# Autodesk Inventor assembly: Flange_tube
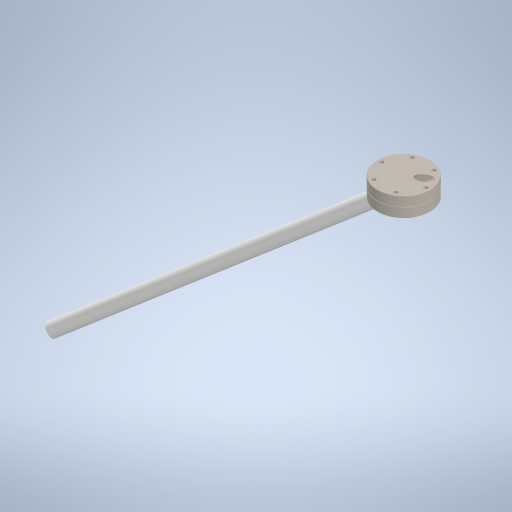
[picture p0: Inventor's stored thumbnail of the model, 512x512]
Saved by Autodesk Inventor 2024 (Build 280153000, 153)
## iProperties
Created: 2024-11-06
Part Number: Flange_tube
Document SubType Name: Assembly
Designer: Andreas Weber
Author: Andreas Weber
## Documents named in this file (4)
- C:\Users\Andreas Weber\Desktop\Upload for Github\Flange_tube.iam
- C:\Users\Andreas Weber\Desktop\Upload for Github\blank_flange_CF40.ipt
- C:\Users\Andreas Weber\Desktop\Upload for Github\blank_flange_thread_CF40.ipt
- C:\Users\Andreas Weber\Desktop\Upload for Github\tube_Brewster_angle.ipt
## Components (3 placed, 3 different names)
1. blank_flange_CF40:1 — Drehbar:1, Verschiebbar:1
2. blank_flange_thread_CF40:1 — Drehbar:1
3. tube_Brewster_angle:1 — Verschiebbar:1
## Relationships (2: RevoluteJoint 1, TranslationJoint 1)
- Drehbar:1 [RevoluteJoint]: blank_flange_CF40:1 ↔ blank_flange_thread_CF40:1
- Verschiebbar:1 [TranslationJoint]: blank_flange_CF40:1 ↔ tube_Brewster_angle:1
